# Autodesk Inventor assembly: ServoWithServoPlate
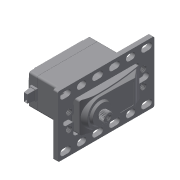
[picture p0: Inventor's stored thumbnail of the model, 180x180]
Saved by Autodesk Inventor 2018 (Build 220112000, 112)
## iProperties
Created: 2018-10-29
Part Number: ServoWithServoPlate
Document SubType Name: Assembly
Designer: ball
Author: ball
## Documents named in this file (3)
- C:\FTC\FTC8863CAD\2018Robot\ServoWithServoPlate.iam
- C:\FTC\FTC8863CAD\GoBilda\1801 Parts\1801-0040-0001.ipt
- C:\FTC\FTC8863CAD\GoBilda\2000 Parts\2000-0025-0001 part.ipt
## Components (2 placed, 2 different names)
1. 1801-0040-0001:1 — Mate:1, Mate:2, Mate:3
2. 2000-0025-0001 part:1 — Mate:1, Mate:2, Mate:3
## Relationships (3: Mate 3)
- Mate:1: 1801-0040-0001:1 ↔ 2000-0025-0001 part:1
- Mate:2: 1801-0040-0001:1 ↔ 2000-0025-0001 part:1
- Mate:3: 1801-0040-0001:1 ↔ 2000-0025-0001 part:1
